# Autodesk Inventor assembly: Double Acting Piston With Hardware
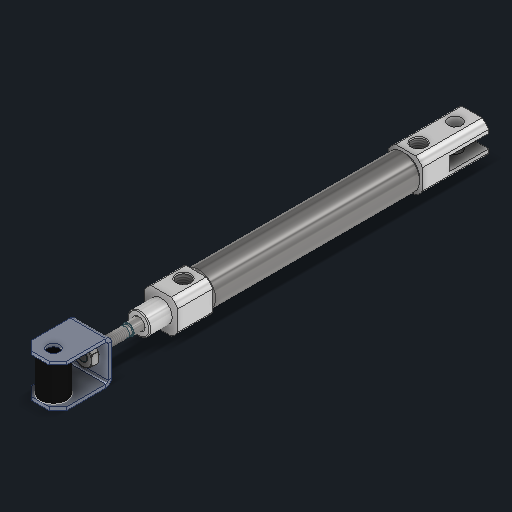
[picture p0: Inventor's stored thumbnail of the model, 512x512]
Saved by Autodesk Inventor 2025.1 (Build 291241000, 241)
## iProperties
Created: 2024-10-23
Part Number: Double Acting Piston With Hardware
Document SubType Name: Assembly
Designer: avere
Author: avere
## Documents named in this file (6)
- C:\Users\avere\VEX\High Stakes\CAD\ROBOPROS-CAD-Inventor\Motion\Pneumatics\Double Acting Piston With Hardware.iam
- C:\Users\avere\VEX\High Stakes\CAD\ROBOPROS-CAD-Inventor\Motion\Pneumatics\Double Acting Piston.iam
- C:\Users\avere\VEX\High Stakes\CAD\ROBOPROS-CAD-Inventor\Motion\Pneumatics\Cylinder Mount.ipt
- C:\Users\avere\VEX\High Stakes\CAD\ROBOPROS-CAD-Inventor\Structure\Hardware\Nut Hex #6-32.ipt
- C:\Users\avere\VEX\High Stakes\CAD\ROBOPROS-CAD-Inventor\Motion\Spacers\Spacer Nylon .375 OD\NSpacer .375 OD x .500.ipt
- C:\Users\avere\VEX\High Stakes\CAD\ROBOPROS-CAD-Inventor\Motion\Spacers\Spacer Nylon .375 OD.ipt
## Components (5 placed, 4 different names)
1. Double Acting Piston:1 [sub-assembly] — Insert:3
2. Cylinder Mount:1 — Insert:1, Insert:2, Insert:4
3. Nut Hex #6-32:1 — Insert:2
4. Nut Hex #6-32:2 — Insert:1, Insert:3
5. NSpacer .375 OD x .500:1 — Insert:4
## Relationships (4: Insert 4)
- Insert:1: Cylinder Mount:1 ↔ Nut Hex #6-32:2
- Insert:2: Cylinder Mount:1 ↔ Nut Hex #6-32:1
- Insert:3: Double Acting Piston:1 ↔ Nut Hex #6-32:2
- Insert:4: Cylinder Mount:1 ↔ NSpacer .375 OD x .500:1
